# Autodesk Inventor assembly: Gear
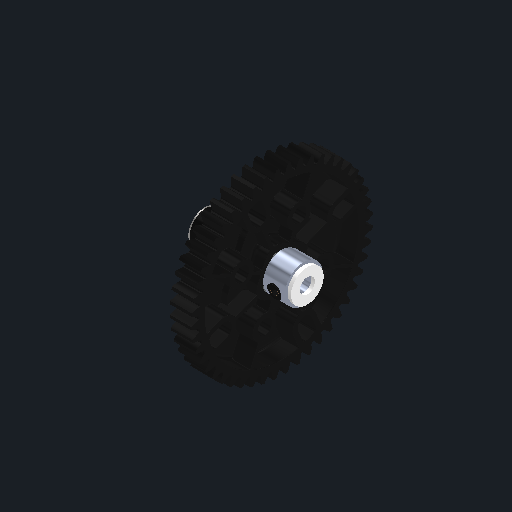
[picture p0: Inventor's stored thumbnail of the model, 512x512]
Saved by Autodesk Inventor 2025 (Build 290162000, 162)
## iProperties
Created: 2024-10-18
Part Number: Gear
Document SubType Name: Assembly
Designer: averey
Author: averey
## Documents named in this file (9)
- D:\VEX\High Stakes\CAD\V2\Chassis\Drivebay Left\Gear.iam
- D:\vex_robotics_high_stakes\hardware\cad\robpros_cad_lib\Motion\Spacers\Washer Steel\SWasher .375 OD x .015625.ipt
- C:\Users\avere\vex_robotics_high_stakes\hardware\cad\robpros_cad_lib\Motion\Spacers\Washer Steel.ipt
- D:\vex_robotics_high_stakes\hardware\cad\robpros_cad_lib\Modified Parts\modified_parts\Half Cut HS 48T Gear, No Insert.ipt
- D:\vex_robotics_high_stakes\hardware\cad\robpros_cad_lib\Motion\Shaft LS\Shaft Collar ipts\Shaft Collar Set Screw.ipt
- D:\vex_robotics_high_stakes\hardware\cad\robpros_cad_lib\Motion\Spacers\Washer Teflon\TWasher .375 OD x .04000.ipt
- C:\Users\avere\vex_robotics_high_stakes\hardware\cad\robpros_cad_lib\Motion\Spacers\Washer Teflon.ipt
- D:\VEX\High Stakes\CAD\ROBOPROS-CAD-Inventor\Motion\Spacers\Spacer Nylon .375 OD\NSpacer .375 OD x .500.ipt
- D:\VEX\High Stakes\CAD\ROBOPROS-CAD-Inventor\Motion\Spacers\Spacer Nylon .375 OD.ipt
## Components (5 placed, 5 different names)
1. Half Cut HS 48T Gear, No Insert:1 — Insert:3
2. Shaft Collar Set Screw:1
3. TWasher .375 OD x .04000:1 — Mate:1
4. SWasher .375 OD x .015625:1 — Insert:4
5. NSpacer .375 OD x .500:1 — Insert:3, Insert:4
## Relationships (5: Insert 4, Mate 1)
- [Insert]: Shaft Collar Set Screw:1 ↔ TWasher .375 OD x .04000:1
- [Insert]: Half Cut HS 48T Gear, No Insert:1 ↔ Shaft Collar Set Screw:1
- Mate:1: TWasher .375 OD x .04000:1
- Insert:3: Half Cut HS 48T Gear, No Insert:1 ↔ NSpacer .375 OD x .500:1
- Insert:4: SWasher .375 OD x .015625:1 ↔ NSpacer .375 OD x .500:1
